# Autodesk Inventor assembly: steelframeparts
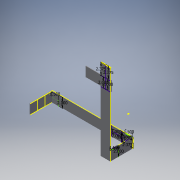
[picture p0: Inventor's stored thumbnail of the model, 180x180]
Saved by Autodesk Inventor 2017 (Build 210142000, 142)
## iProperties
Created: 2017-03-02
Part Number: steelframeparts
Document SubType Name: Assembly
Designer: Jess
Author: Jess
## Documents named in this file (7)
- C:\Users\Jess\Documents\Parts for new robot\pickup\steelframeparts.iam
- C:\Users\Jess\Documents\Parts for new robot\pickup\long metal piece 2x17.ipt
- C:\Users\Jess\Documents\Parts for new robot\pickup\short top side 5.25x2.ipt
- C:\Users\Jess\Documents\Parts for new robot\pickup\bottom near wheel 4.5x2.ipt
- C:\Users\Jess\Documents\Parts for new robot\pickup\corner piece 2x1.5.ipt
- C:\Users\Jess\Documents\Parts for new robot\pickup\bottom near wheel 4.5x2_MIR.ipt
- C:\Users\Jess\Documents\Parts for new robot\pickup\corner piece 2x1.5_MIR.ipt
## Components (7 placed, 6 different names)
1. long metal piece 2x17:2 — Mate:2, Mate:5, Mate:21, Mate:22
2. long metal piece 2x17:3 — Mate:16, Mate:17, Mate:18, Mate:19, Mate:20
3. short top side 5.25x2:2 — Mate:2, Mate:5
4. bottom near wheel 4.5x2:2 — Mate:7, Mate:8, Mate:9, Mate:18, Mate:21, Mate:22
5. corner piece 2x1.5:3 — Mate:7, Mate:8, Mate:9, Mate:16, Mate:17
6. bottom near wheel 4.5x2_MIR:1 — Mate:13, Mate:14, Mate:15, Mate:20
7. corner piece 2x1.5_MIR:1 — Mate:13, Mate:14, Mate:15, Mate:19
## Relationships (15: Mate 15)
- Mate:2: long metal piece 2x17:2 ↔ short top side 5.25x2:2
- Mate:5: long metal piece 2x17:2 ↔ short top side 5.25x2:2
- Mate:7: bottom near wheel 4.5x2:2 ↔ corner piece 2x1.5:3
- Mate:8: bottom near wheel 4.5x2:2 ↔ corner piece 2x1.5:3
- Mate:9: bottom near wheel 4.5x2:2 ↔ corner piece 2x1.5:3
- Mate:13: bottom near wheel 4.5x2_MIR:1 ↔ corner piece 2x1.5_MIR:1
- Mate:14: bottom near wheel 4.5x2_MIR:1 ↔ corner piece 2x1.5_MIR:1
- Mate:15: bottom near wheel 4.5x2_MIR:1 ↔ corner piece 2x1.5_MIR:1
- Mate:16: long metal piece 2x17:3 ↔ corner piece 2x1.5:3
- Mate:17: long metal piece 2x17:3 ↔ corner piece 2x1.5:3
- Mate:18: long metal piece 2x17:3 ↔ bottom near wheel 4.5x2:2
- Mate:19: long metal piece 2x17:3 ↔ corner piece 2x1.5_MIR:1
- Mate:20: long metal piece 2x17:3 ↔ bottom near wheel 4.5x2_MIR:1
- Mate:21: long metal piece 2x17:2 ↔ bottom near wheel 4.5x2:2
- Mate:22: long metal piece 2x17:2 ↔ bottom near wheel 4.5x2:2
